# Autodesk Inventor assembly: TopAndIntermediaryAxle
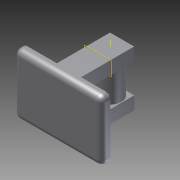
[picture p0: Inventor's stored thumbnail of the model, 180x180]
Saved by Autodesk Inventor 2012 (Build 160160000, 160)
## iProperties
Created: 2011-11-03
Part Number: TopAndIntermediaryAxle
Document SubType Name: Assembly
Designer: Drew
Author: Drew
## Documents named in this file (4)
- C:\Users\Drew\Dropbox\Hexapod Research\Leg Design\Other Parts\Intermediary Gear Box\Assemblies\TopAndIntermediaryAxle.iam
- C:\Users\Drew\Dropbox\Hexapod Research\Leg Design\Other Parts\Intermediary Gear Box\GearBoxTop.ipt
- C:\Users\Drew\Dropbox\Hexapod Research\Leg Design\Other Parts\Intermediary Gear Box\LargeSmallGearAxis.ipt
- C:\Users\Drew\Dropbox\Hexapod Research\Leg Design\Other Parts\Intermediary Gear Box\DerivedPartsFromAssemblies\TransferGear.ipt
## Components (3 placed, 3 different names)
1. GearBoxTop:1 — Flush:3, Flush:4, Flush:5
2. LargeSmallGearAxis:1 — Flush:3, Mate:2, Mate:3, Flush:4, Flush:5
3. TransferGear:1 — Mate:2, Mate:3
## Relationships (5: Flush 3, Mate 2)
- Flush:3: GearBoxTop:1 ↔ LargeSmallGearAxis:1
- Mate:2: LargeSmallGearAxis:1 ↔ TransferGear:1
- Mate:3 (0.3 mm): LargeSmallGearAxis:1 ↔ TransferGear:1
- Flush:4: GearBoxTop:1 ↔ LargeSmallGearAxis:1
- Flush:5: GearBoxTop:1 ↔ LargeSmallGearAxis:1
